# Autodesk Inventor assembly: XCarriage90
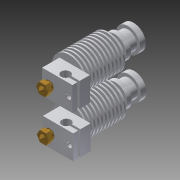
[picture p0: Inventor's stored thumbnail of the model, 180x180]
Saved by Autodesk Inventor 2015 (Build 190159000, 159)
## iProperties
Created: 2014-10-04
Part Number: XCarriage90
Document SubType Name: Assembly
Designer: Jack
Author: Jack
## Documents named in this file (2)
- C:\Users\Jack\ownCloud\Projects\CoreXY\InventorModel\XAxis\XCarriage90.iam
- C:\Users\Jack\ownCloud\Projects\CoreXY\InventorModel\Extruder\E3DV6\E3DV6.iam
## Components (2 placed, 1 different names)
1. E3DV6:1 [sub-assembly] — Angle:1, Flush:1, Angle:3
2. E3DV6:2 [sub-assembly] — Angle:2, Flush:1, Angle:4
## Relationships (5: Angle 4, Flush 1)
- Angle:1 (180 deg): E3DV6:1
- Angle:2 (180 deg): E3DV6:2
- Flush:1: E3DV6:1 ↔ E3DV6:2
- Angle:3 (180 deg): E3DV6:1
- Angle:4 (0 deg): E3DV6:2
